# Autodesk Inventor assembly: 217-3433-PTO Config STEP
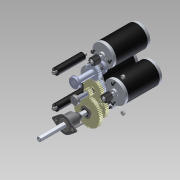
[picture p0: Inventor's stored thumbnail of the model, 180x180]
Saved by Autodesk Inventor 2015 (Build 190159000, 159)
## iProperties
Created: 2015-12-15
Part Number: 217-3433-PTO Config STEP
Document SubType Name: Assembly
Designer: Daniel
Title: 217-3433-PTO Config STEP.STEP
Description: STEP AP214
Creation Date: 2013-12-10
Sending System: SolidWorks 2013
Preprocessor: SwSTEP 2.0
Author: Daniel
## Documents named in this file (45)
- C:\Users\Daniel\Documents\Inventor\West Coast Drive\Imported Components\WCD gear box\217-3433 WCD gear box assembly.iam
- C:\Users\Daniel\Documents\Inventor\West Coast Drive\Imported Components\WCD gear box\217-2428-027 Rev1_97414A630.ipt
- C:\Users\Daniel\Documents\Inventor\West Coast Drive\Imported Components\WCD gear box\217-3423-005 Rev1.ipt
- C:\Users\Daniel\Documents\Inventor\West Coast Drive\Imported Components\WCD gear box\217-3195-200 Rev1.iam
- C:\Users\Daniel\Documents\Inventor\West Coast Drive\Imported Components\WCD gear box\217-3489.ipt
- C:\Users\Daniel\Documents\Inventor\West Coast Drive\Imported Components\WCD gear box\217-3423-006 Rev1.ipt
- C:\Users\Daniel\Documents\Inventor\West Coast Drive\Imported Components\WCD gear box\217-3423-008 Rev1.ipt
- C:\Users\Daniel\Documents\Inventor\West Coast Drive\Imported Components\WCD gear box\217-3423-009 Rev1.ipt
- C:\Users\Daniel\Documents\Inventor\West Coast Drive\Imported Components\WCD gear box\217-2778-001 Rev2_NCQ8A075-050M.iam
- C:\Users\Daniel\Documents\Inventor\West Coast Drive\Imported Components\WCD gear box\217-2731.ipt
- C:\Users\Daniel\Documents\Inventor\West Coast Drive\Imported Components\WCD gear box\217-2733.ipt
- C:\Users\Daniel\Documents\Inventor\West Coast Drive\Imported Components\WCD gear box\217-2734.ipt
- C:\Users\Daniel\Documents\Inventor\West Coast Drive\Imported Components\WCD gear box\217-2743.ipt
- C:\Users\Daniel\Documents\Inventor\West Coast Drive\Imported Components\WCD gear box\217-2614-002_98430A132.ipt
- C:\Users\Daniel\Documents\Inventor\West Coast Drive\Imported Components\WCD gear box\217-3421-007 Rev1.ipt
- C:\Users\Daniel\Documents\Inventor\West Coast Drive\Imported Components\WCD gear box\217-3421-009 Rev1.ipt
- C:\Users\Daniel\Documents\Inventor\West Coast Drive\Imported Components\WCD gear box\217-3421-010 Rev1.ipt
- C:\Users\Daniel\Documents\Inventor\West Coast Drive\Imported Components\WCD gear box\217-3421-011 Rev2_97633A200.ipt
- C:\Users\Daniel\Documents\Inventor\West Coast Drive\Imported Components\WCD gear box\217-3422-007 Rev1.ipt
- C:\Users\Daniel\Documents\Inventor\West Coast Drive\Imported Components\WCD gear box\217-3423-014 Rev1.ipt
- C:\Users\Daniel\Documents\Inventor\West Coast Drive\Imported Components\WCD gear box\217-3423-016 Rev1.ipt
- C:\Users\Daniel\Documents\Inventor\West Coast Drive\Imported Components\WCD gear box\217-3424-003 Rev1.ipt
- C:\Users\Daniel\Documents\Inventor\West Coast Drive\Imported Components\WCD gear box\217-3210-001 Rev1_30t.ipt
- C:\Users\Daniel\Documents\Inventor\West Coast Drive\Imported Components\WCD gear box\217-3215-001 Rev1_42t.ipt
- C:\Users\Daniel\Documents\Inventor\West Coast Drive\Imported Components\WCD gear box\217-3414-001 Rev1_14t Steel Pinion.ipt
- C:\Users\Daniel\Documents\Inventor\West Coast Drive\Imported Components\WCD gear box\217-3418-001 Rev2_44t.ipt
- C:\Users\Daniel\Documents\Inventor\West Coast Drive\Imported Components\WCD gear box\217-3420-001 Rev2_60t.ipt
- C:\Users\Daniel\Documents\Inventor\West Coast Drive\Imported Components\WCD gear box\217-3100-001_14t.ipt
- C:\Users\Daniel\Documents\Inventor\West Coast Drive\Imported Components\WCD gear box\217-2000.ipt
- C:\Users\Daniel\Documents\Inventor\West Coast Drive\Imported Components\WCD gear box\217-3433-001 Rev1_Default_As Machined_.ipt
- C:\Users\Daniel\Documents\Inventor\West Coast Drive\Imported Components\WCD gear box\217-3423-003 Rev1.ipt
- C:\Users\Daniel\Documents\Inventor\West Coast Drive\Imported Components\WCD gear box\217-3424-005 Rev1.ipt
- C:\Users\Daniel\Documents\Inventor\West Coast Drive\Imported Components\WCD gear box\217-3256-001 Rev1.ipt
- C:\Users\Daniel\Documents\Inventor\West Coast Drive\Imported Components\WCD gear box\217-3257-001 Rev1.ipt
- C:\Users\Daniel\Documents\Inventor\West Coast Drive\Imported Components\WCD gear box\217-3259-001 Rev1.ipt
- C:\Users\Daniel\Documents\Inventor\West Coast Drive\Imported Components\WCD gear box\217-3423-004 Rev1.ipt
- C:\Users\Daniel\Documents\Inventor\West Coast Drive\Imported Components\WCD gear box\217-3424-002 Rev1.ipt
- C:\Users\Daniel\Documents\Inventor\West Coast Drive\Imported Components\WCD gear box\217-2758-001 Rev1.ipt
- C:\Users\Daniel\Documents\Inventor\West Coast Drive\Imported Components\WCD gear box\217-3422-004 Rev2.ipt
- C:\Users\Daniel\Documents\Inventor\West Coast Drive\Imported Components\WCD gear box\217-3263-001 Rev1.ipt
- C:\Users\Daniel\Documents\Inventor\West Coast Drive\Imported Components\WCD gear box\217-2761-001 rev1.ipt
- C:\Users\Daniel\Documents\Inventor\West Coast Drive\Imported Components\217-3433-STEP\217-3433-003 Rev1.ipt
- C:\Users\Daniel\Documents\Inventor\West Coast Drive\Imported Components\217-3433-STEP\217-2705-001_30t.ipt
- C:\Users\Daniel\Documents\Inventor\West Coast Drive\Imported Components\217-3433-STEP\217-3261-001 Rev1.ipt
- C:\Users\Daniel\Documents\Inventor\West Coast Drive\Imported Components\217-3433-STEP\217-2731.ipt
## Components (78 placed, 78 different names)
1. 217-2428-027 Rev1_97414A630_1 — Mate:126, Mate:127
2. 217-3423-005 Rev1_2 — Mate:106, Mate:108, Mate:109, Mate:110, Mate:111, Mate:112, Mate:113, Mate:114, Angle:4
3. 217-3195-200 Rev1_3 [sub-assembly] — Mate:128, Angle:6, Mate:129, Mate:130
4. 217-3489_4 — Mate:124, Mate:125, Mate:127, Mate:130
5. 217-3423-006 Rev1_9 — Mate:107, Mate:108
6. 217-3423-006 Rev1_10 — Mate:105, Mate:106, Mate:117
7. 217-3423-008 Rev1_11 — Mate:102, Mate:103, Mate:124, Mate:125, Mate:126, Mate:167
8. 217-3423-009 Rev1_13 — Mate:164, Mate:165, Mate:166, Angle:14
9. 217-2778-001 Rev2_NCQ8A075-050M_16 [sub-assembly] — Mate:113, Mate:114, Angle:4, Mate:128, Angle:6, Mate:129
10. 217-2731_17 — Mate:101, Mate:120, Mate:121, Mate:122, Mate:134, Mate:135, Mate:136
11. 217-2731_18 — Mate:151, Mate:153, Mate:156, Mate:157, Flush:8
12. 217-2733_19 — Flush:7, Mate:140, Mate:148, Mate:149, Mate:150
13. 217-2733_20 — Flush:6, Mate:139
14. 217-2734_21 — Mate:79, Mate:89, Mate:90, Angle:13
15. 217-2734_23 — Mate:91, Mate:92, Mate:93, Mate:94, Angle:2
16. 217-2743_24 — Mate:100, Mate:101, Mate:102, Mate:118, Mate:123, Mate:163
17. 217-2614-002_98430A132_26 — Mate:18, Mate:19
18. 217-2614-002_98430A132_27 — Mate:20, Mate:21
19. 217-2614-002_98430A132_28 — Mate:37, Mate:38
20. 217-2614-002_98430A132_29 — Mate:35, Mate:36
21. 217-2614-002_98430A132_30 — Mate:9, Mate:12
22. 217-2614-002_98430A132_31 — Mate:10, Mate:11
23. 217-3421-007 Rev1_34 — Mate:105, Mate:110, Mate:111, Mate:116
24. 217-3421-007 Rev1_35 — Mate:107, Mate:109, Mate:112, Mate:115
25. 217-3421-009 Rev1_36 — Mate:4, Mate:5
26. 217-3421-009 Rev1_37 — Mate:29, Mate:30
27. 217-3421-009 Rev1_38 — Mate:6, Mate:7
28. 217-3421-009 Rev1_39 — Mate:44, Mate:45
29. 217-3421-009 Rev1_40 — Mate:43, Mate:46
30. 217-3421-009 Rev1_41 — Mate:27, Mate:28
31. 217-3421-010 Rev1_42 — Mate:60, Mate:61
32. 217-3421-010 Rev1_43 — Mate:72, Mate:73
33. 217-3421-010 Rev1_44 — Mate:64, Mate:65
34. 217-3421-010 Rev1_45 — Mate:68, Mate:69
35. 217-3421-011 Rev2_97633A200_47 — Mate:168, Mate:169
36. 217-3422-007 Rev1_48 — Mate:75, Flush:2, Mate:76
37. 217-3422-007 Rev1_49 — Mate:74, Flush:1, Mate:77
38. 217-3423-014 Rev1_50 — Mate:164, Mate:165, Mate:167
39. 217-3423-016 Rev1_52 — Mate:131, Mate:136
40. 217-3423-016 Rev1_53 — Mate:133, Mate:135
41. 217-3423-016 Rev1_54 — Mate:132, Mate:134
42. 217-3424-003 Rev1_55 — Mate:70, Mate:71, Mate:72
43. 217-3424-003 Rev1_56 — Mate:66, Mate:67, Mate:68
44. 217-3424-003 Rev1_57 — Mate:62, Mate:63, Mate:64
45. 217-3424-003 Rev1_58 — Mate:58, Mate:59, Mate:60
46. 217-3210-001 Rev1_30t_59 — Mate:143, Mate:147, Angle:10, Mate:148, Rotation:6
47. 217-3215-001 Rev1_42t_60 — Mate:141, Mate:143, Mate:146, Angle:9, Angle:10, Rotation:2, Rotation:4, Rotation:5
48. 217-3414-001 Rev1_14t Steel Pinion_61 — Mate:34, Mate:36, Mate:37, Mate:39, Rotation:5
49. 217-3414-001 Rev1_14t Steel Pinion_62 — Mate:17, Mate:19, Mate:21, Mate:22, Rotation:4
50. 217-3414-001 Rev1_14t Steel Pinion_63 — Mate:8, Mate:9, Mate:10, Mate:13, Rotation:3
51. 217-3418-001 Rev2_44t_64 — Mate:103, Mate:118, Rotation:6
52. 217-3420-001 Rev2_60t_65 — Mate:91, Mate:92, Mate:96, Angle:14, Angle:15, Rotation:1
53. 217-3100-001_14t_66 — Mate:142, Mate:144, Angle:7, Angle:8, Rotation:1
54. 217-2000_68 — Mate:14, Mate:15, Mate:16, Mate:17, Mate:18, Mate:20, Mate:22, Mate:23, Mate:25, Mate:26
55. 217-2000_69 — Mate:31, Mate:32, Mate:33, Mate:34, Mate:35, Mate:38, Mate:39, Mate:40, Mate:41, Mate:42
56. 217-2000_70 — Mate:1, Mate:2, Mate:3, Mate:8, Mate:11, Mate:12, Mate:13
57. 217-3433-001 Rev1_Default<As Machined>_71 — Mate:1, Mate:2, Mate:3, Mate:4, Mate:5, Mate:6, Mate:7, Mate:23, Mate:25, Mate:26, Mate:27, Mate:28, Mate:29, Mate:30, Mate:40, Mate:41, Mate:42, Mate:43, Mate:44, Mate:45, Mate:46, Mate:47, Mate:48, Mate:49, Mate:50, Mate:51, Mate:52, Mate:53, Mate:54, Mate:61, Mate:65, Mate:69, Mate:73, Mate:88, Mate:115, Mate:116, Mate:117, Mate:120, Mate:121, Mate:131, Mate:132, Mate:133, Mate:149, Mate:150, Mate:154, Mate:155
58. 217-3433-001 Rev1_Default<As Machined>_72 — Mate:55, Mate:56, Mate:57, Mate:58, Mate:59, Mate:63, Mate:67, Mate:71, Mate:76, Mate:77, Mate:78, Mate:151, Mate:156
59. 217-3423-003 Rev1_73 — Mate:87, Angle:1, Mate:88, Mate:96, Mate:163, Mate:166, Mate:168, Mate:169, Angle:13, Angle:15
60. 217-3424-005 Rev1_75 — Flush:6, Mate:139, Flush:7, Mate:140, Mate:144, Mate:145, Mate:146, Mate:147, Angle:7
61. 217-3256-001 Rev1_76 — Mate:141, Mate:142, Mate:145, Angle:8, Angle:9
62. 217-3257-001 Rev1_78 — Mate:93, Mate:94, Angle:2, Mate:95
63. 217-3423-004 Rev1_81 — Mate:100, Mate:122, Mate:123
64. 217-3424-002 Rev1_84 — Mate:49, Mate:50, Mate:66
65. 217-3424-002 Rev1_85 — Mate:52, Mate:54, Mate:56, Mate:70
66. 217-3424-002 Rev1_86 — Mate:47, Mate:48, Mate:62
67. 217-3424-002 Rev1_87 — Mate:51, Mate:53, Mate:55, Mate:57
68. 217-3422-004 Rev2_89 — Mate:74, Flush:1, Mate:75, Flush:2, Mate:78, Mate:79, Mate:90
69. 217-3263-001 Rev1_91 — Mate:81, Mate:82, Mate:83, Mate:86, Flush:3, Mate:87, Angle:1, Mate:89
70. 217-3259-001 Rev1_92 — Mate:81, Mate:85, Mate:86, Flush:3, Flush:4
71. 217-2758-001 Rev1_93 — Mate:83, Mate:84, Flush:5, Mate:95
72. 217-2761-001 rev1_94 — Mate:14, Mate:15, Mate:16
73. 217-2761-001 rev1_95 — Mate:31, Mate:32, Mate:33
74. 217-3257-001 Rev1_100 — Mate:82, Mate:84, Mate:85, Flush:4, Flush:5
75. 217-3433-003 Rev1:1 — Mate:153, Mate:157, Flush:8, Mate:158, Mate:159, Angle:11, Angle:12
76. 217-2705-001_30t:1 — Mate:158, Angle:12, Mate:160, Rotation:2, Rotation:3
77. 217-3261-001 Rev1:1 — Mate:159, Angle:11, Mate:160, Mate:161
78. 217-2731:3 — Mate:154, Mate:155, Mate:161
## Relationships (185: Mate 158, Angle 13, Flush 8, RelateRotation 6)
- Mate:1: 217-2000_70 ↔ 217-3433-001 Rev1_Default<As Machined>_71
- Mate:2: 217-2000_70 ↔ 217-3433-001 Rev1_Default<As Machined>_71
- Mate:3: 217-2000_70 ↔ 217-3433-001 Rev1_Default<As Machined>_71
- Mate:4: 217-3421-009 Rev1_36 ↔ 217-3433-001 Rev1_Default<As Machined>_71
- Mate:5: 217-3421-009 Rev1_36 ↔ 217-3433-001 Rev1_Default<As Machined>_71
- Mate:6: 217-3421-009 Rev1_38 ↔ 217-3433-001 Rev1_Default<As Machined>_71
- Mate:7: 217-3421-009 Rev1_38 ↔ 217-3433-001 Rev1_Default<As Machined>_71
- Mate:8: 217-3414-001 Rev1_14t Steel Pinion_63 ↔ 217-2000_70
- Mate:9: 217-2614-002_98430A132_30 ↔ 217-3414-001 Rev1_14t Steel Pinion_63
- Mate:10: 217-2614-002_98430A132_31 ↔ 217-3414-001 Rev1_14t Steel Pinion_63
- Mate:11: 217-2614-002_98430A132_31 ↔ 217-2000_70
- Mate:12: 217-2614-002_98430A132_30 ↔ 217-2000_70
- Mate:13 (10.2113 mm): 217-3414-001 Rev1_14t Steel Pinion_63 ↔ 217-2000_70
- Mate:14: 217-2000_68 ↔ 217-2761-001 rev1_94
- Mate:15: 217-2000_68 ↔ 217-2761-001 rev1_94
- Mate:16: 217-2000_68 ↔ 217-2761-001 rev1_94
- Mate:17: 217-3414-001 Rev1_14t Steel Pinion_62 ↔ 217-2000_68
- Mate:18: 217-2614-002_98430A132_26 ↔ 217-2000_68
- Mate:19: 217-2614-002_98430A132_26 ↔ 217-3414-001 Rev1_14t Steel Pinion_62
- Mate:20: 217-2614-002_98430A132_27 ↔ 217-2000_68
- Mate:21: 217-2614-002_98430A132_27 ↔ 217-3414-001 Rev1_14t Steel Pinion_62
- Mate:22 (10.2113 mm): 217-3414-001 Rev1_14t Steel Pinion_62 ↔ 217-2000_68
- Mate:23: 217-2000_68 ↔ 217-3433-001 Rev1_Default<As Machined>_71
- Mate:25: 217-2000_68 ↔ 217-3433-001 Rev1_Default<As Machined>_71
- Mate:26: 217-2000_68 ↔ 217-3433-001 Rev1_Default<As Machined>_71
- Mate:27: 217-3421-009 Rev1_41 ↔ 217-3433-001 Rev1_Default<As Machined>_71
- Mate:28: 217-3421-009 Rev1_41 ↔ 217-3433-001 Rev1_Default<As Machined>_71
- Mate:29: 217-3421-009 Rev1_37 ↔ 217-3433-001 Rev1_Default<As Machined>_71
- Mate:30: 217-3421-009 Rev1_37 ↔ 217-3433-001 Rev1_Default<As Machined>_71
- Mate:31: 217-2000_69 ↔ 217-2761-001 rev1_95
- Mate:32: 217-2000_69 ↔ 217-2761-001 rev1_95
- Mate:33: 217-2000_69 ↔ 217-2761-001 rev1_95
- Mate:34: 217-3414-001 Rev1_14t Steel Pinion_61 ↔ 217-2000_69
- Mate:35: 217-2614-002_98430A132_29 ↔ 217-2000_69
- Mate:36: 217-2614-002_98430A132_29 ↔ 217-3414-001 Rev1_14t Steel Pinion_61
- Mate:37: 217-2614-002_98430A132_28 ↔ 217-3414-001 Rev1_14t Steel Pinion_61
- Mate:38: 217-2614-002_98430A132_28 ↔ 217-2000_69
- Mate:39 (10.2113 mm): 217-3414-001 Rev1_14t Steel Pinion_61 ↔ 217-2000_69
- Mate:40: 217-2000_69 ↔ 217-3433-001 Rev1_Default<As Machined>_71
- Mate:41: 217-2000_69 ↔ 217-3433-001 Rev1_Default<As Machined>_71
- Mate:42: 217-2000_69 ↔ 217-3433-001 Rev1_Default<As Machined>_71
- Mate:43: 217-3421-009 Rev1_40 ↔ 217-3433-001 Rev1_Default<As Machined>_71
- Mate:44: 217-3421-009 Rev1_39 ↔ 217-3433-001 Rev1_Default<As Machined>_71
- Mate:45: 217-3421-009 Rev1_39 ↔ 217-3433-001 Rev1_Default<As Machined>_71
- Mate:46: 217-3421-009 Rev1_40 ↔ 217-3433-001 Rev1_Default<As Machined>_71
- Mate:47: 217-3433-001 Rev1_Default<As Machined>_71 ↔ 217-3424-002 Rev1_86
- Mate:48: 217-3433-001 Rev1_Default<As Machined>_71 ↔ 217-3424-002 Rev1_86
- Mate:49: 217-3433-001 Rev1_Default<As Machined>_71 ↔ 217-3424-002 Rev1_84
- Mate:50: 217-3433-001 Rev1_Default<As Machined>_71 ↔ 217-3424-002 Rev1_84
- Mate:51: 217-3433-001 Rev1_Default<As Machined>_71 ↔ 217-3424-002 Rev1_87
- Mate:52: 217-3433-001 Rev1_Default<As Machined>_71 ↔ 217-3424-002 Rev1_85
- Mate:53: 217-3433-001 Rev1_Default<As Machined>_71 ↔ 217-3424-002 Rev1_87
- Mate:54: 217-3433-001 Rev1_Default<As Machined>_71 ↔ 217-3424-002 Rev1_85
- Mate:55: 217-3433-001 Rev1_Default<As Machined>_72 ↔ 217-3424-002 Rev1_87
- Mate:56: 217-3433-001 Rev1_Default<As Machined>_72 ↔ 217-3424-002 Rev1_85
- Mate:57: 217-3433-001 Rev1_Default<As Machined>_72 ↔ 217-3424-002 Rev1_87
- Mate:58: 217-3424-003 Rev1_58 ↔ 217-3433-001 Rev1_Default<As Machined>_72
- Mate:59: 217-3424-003 Rev1_58 ↔ 217-3433-001 Rev1_Default<As Machined>_72
- Mate:60: 217-3421-010 Rev1_42 ↔ 217-3424-003 Rev1_58
- Mate:61: 217-3421-010 Rev1_42 ↔ 217-3433-001 Rev1_Default<As Machined>_71
- Mate:62: 217-3424-003 Rev1_57 ↔ 217-3424-002 Rev1_86
- Mate:63: 217-3424-003 Rev1_57 ↔ 217-3433-001 Rev1_Default<As Machined>_72
- Mate:64: 217-3421-010 Rev1_44 ↔ 217-3424-003 Rev1_57
- Mate:65: 217-3421-010 Rev1_44 ↔ 217-3433-001 Rev1_Default<As Machined>_71
- Mate:66: 217-3424-003 Rev1_56 ↔ 217-3424-002 Rev1_84
- Mate:67: 217-3424-003 Rev1_56 ↔ 217-3433-001 Rev1_Default<As Machined>_72
- Mate:68: 217-3421-010 Rev1_45 ↔ 217-3424-003 Rev1_56
- Mate:69: 217-3421-010 Rev1_45 ↔ 217-3433-001 Rev1_Default<As Machined>_71
- Mate:70: 217-3424-003 Rev1_55 ↔ 217-3424-002 Rev1_85
- Mate:71: 217-3424-003 Rev1_55 ↔ 217-3433-001 Rev1_Default<As Machined>_72
- Mate:72: 217-3421-010 Rev1_43 ↔ 217-3424-003 Rev1_55
- Mate:73: 217-3421-010 Rev1_43 ↔ 217-3433-001 Rev1_Default<As Machined>_71
- Mate:74: 217-3422-007 Rev1_49 ↔ 217-3422-004 Rev2_89
- Flush:1: 217-3422-007 Rev1_49 ↔ 217-3422-004 Rev2_89
- Mate:75: 217-3422-007 Rev1_48 ↔ 217-3422-004 Rev2_89
- Flush:2: 217-3422-007 Rev1_48 ↔ 217-3422-004 Rev2_89
- Mate:76: 217-3422-007 Rev1_48 ↔ 217-3433-001 Rev1_Default<As Machined>_72
- Mate:77: 217-3422-007 Rev1_49 ↔ 217-3433-001 Rev1_Default<As Machined>_72
- Mate:78: 217-3433-001 Rev1_Default<As Machined>_72 ↔ 217-3422-004 Rev2_89
- Mate:79: 217-2734_21 ↔ 217-3422-004 Rev2_89
- Mate:81: 217-3263-001 Rev1_91 ↔ 217-3259-001 Rev1_92
- Mate:82: 217-3263-001 Rev1_91 ↔ 217-3257-001 Rev1_100
- Mate:83: 217-3263-001 Rev1_91 ↔ 217-2758-001 Rev1_93
- Mate:84: 217-2758-001 Rev1_93 ↔ 217-3257-001 Rev1_100
- Mate:85: 217-3259-001 Rev1_92 ↔ 217-3257-001 Rev1_100
- Mate:86: 217-3263-001 Rev1_91 ↔ 217-3259-001 Rev1_92
- Flush:3: 217-3263-001 Rev1_91 ↔ 217-3259-001 Rev1_92
- Flush:4: 217-3259-001 Rev1_92 ↔ 217-3257-001 Rev1_100
- Flush:5: 217-2758-001 Rev1_93 ↔ 217-3257-001 Rev1_100
- Mate:87: 217-3423-003 Rev1_73 ↔ 217-3263-001 Rev1_91
- Angle:1 (0 deg): 217-3423-003 Rev1_73 ↔ 217-3263-001 Rev1_91
- Mate:88: 217-3433-001 Rev1_Default<As Machined>_71 ↔ 217-3423-003 Rev1_73
- Mate:89: 217-2734_21 ↔ 217-3263-001 Rev1_91
- Mate:90: 217-2734_21 ↔ 217-3422-004 Rev2_89
- Mate:91: 217-2734_23 ↔ 217-3420-001 Rev2_60t_65
- Mate:92: 217-2734_23 ↔ 217-3420-001 Rev2_60t_65
- Mate:93: 217-2734_23 ↔ 217-3257-001 Rev1_78
- Mate:94: 217-2734_23 ↔ 217-3257-001 Rev1_78
- Angle:2 (0 deg): 217-2734_23 ↔ 217-3257-001 Rev1_78
- Mate:95 (18.3389 mm): 217-3257-001 Rev1_78 ↔ 217-2758-001 Rev1_93
- Mate:96: 217-3420-001 Rev2_60t_65 ↔ 217-3423-003 Rev1_73
- Mate:100: 217-2743_24 ↔ 217-3423-004 Rev1_81
- Mate:101: 217-2731_17 ↔ 217-2743_24
- Mate:102: 217-3423-008 Rev1_11 ↔ 217-2743_24
- Mate:103: 217-3423-008 Rev1_11 ↔ 217-3418-001 Rev2_44t_64
- Mate:105: 217-3423-006 Rev1_10 ↔ 217-3421-007 Rev1_34
- Mate:106: 217-3423-005 Rev1_2 ↔ 217-3423-006 Rev1_10
- Mate:107: 217-3423-006 Rev1_9 ↔ 217-3421-007 Rev1_35
- Mate:108: 217-3423-005 Rev1_2 ↔ 217-3423-006 Rev1_9
- Mate:109: 217-3423-005 Rev1_2 ↔ 217-3421-007 Rev1_35
- Mate:110: 217-3423-005 Rev1_2 ↔ 217-3421-007 Rev1_34
- Mate:111: 217-3423-005 Rev1_2 ↔ 217-3421-007 Rev1_34
- Mate:112: 217-3423-005 Rev1_2 ↔ 217-3421-007 Rev1_35
- Mate:113: 217-3423-005 Rev1_2 ↔ 217-2778-001 Rev2_NCQ8A075-050M_16
- Mate:114: 217-3423-005 Rev1_2 ↔ 217-2778-001 Rev2_NCQ8A075-050M_16
- Mate:115: 217-3421-007 Rev1_35 ↔ 217-3433-001 Rev1_Default<As Machined>_71
- Mate:116: 217-3421-007 Rev1_34 ↔ 217-3433-001 Rev1_Default<As Machined>_71
- Mate:117: 217-3423-006 Rev1_10 ↔ 217-3433-001 Rev1_Default<As Machined>_71
- Angle:4 (1.1459 deg): 217-3423-005 Rev1_2 ↔ 217-2778-001 Rev2_NCQ8A075-050M_16
- Mate:118: 217-2743_24 ↔ 217-3418-001 Rev2_44t_64
- Mate:120: 217-2731_17 ↔ 217-3433-001 Rev1_Default<As Machined>_71
- Mate:121: 217-2731_17 ↔ 217-3433-001 Rev1_Default<As Machined>_71
- Mate:122: 217-2731_17 ↔ 217-3423-004 Rev1_81
- Mate:123: 217-2743_24 ↔ 217-3423-004 Rev1_81
- Mate:124: 217-3489_4 ↔ 217-3423-008 Rev1_11
- Mate:125: 217-3489_4 ↔ 217-3423-008 Rev1_11
- Mate:126: 217-2428-027 Rev1_97414A630_1 ↔ 217-3423-008 Rev1_11
- Mate:127: 217-2428-027 Rev1_97414A630_1 ↔ 217-3489_4
- Mate:128: 217-3195-200 Rev1_3 ↔ 217-2778-001 Rev2_NCQ8A075-050M_16
- Angle:6 (180 deg): 217-3195-200 Rev1_3 ↔ 217-2778-001 Rev2_NCQ8A075-050M_16
- Mate:129: 217-3195-200 Rev1_3 ↔ 217-2778-001 Rev2_NCQ8A075-050M_16
- Mate:130: 217-3195-200 Rev1_3 ↔ 217-3489_4
- Mate:131: 217-3423-016 Rev1_52 ↔ 217-3433-001 Rev1_Default<As Machined>_71
- Mate:132: 217-3423-016 Rev1_54 ↔ 217-3433-001 Rev1_Default<As Machined>_71
- Mate:133: 217-3423-016 Rev1_53 ↔ 217-3433-001 Rev1_Default<As Machined>_71
- Mate:134: 217-2731_17 ↔ 217-3423-016 Rev1_54
- Mate:135: 217-2731_17 ↔ 217-3423-016 Rev1_53
- Mate:136: 217-2731_17 ↔ 217-3423-016 Rev1_52
- Flush:6: 217-2733_20 ↔ 217-3424-005 Rev1_75
- Mate:139: 217-2733_20 ↔ 217-3424-005 Rev1_75
- Flush:7: 217-2733_19 ↔ 217-3424-005 Rev1_75
- Mate:140: 217-2733_19 ↔ 217-3424-005 Rev1_75
- Mate:141: 217-3215-001 Rev1_42t_60 ↔ 217-3256-001 Rev1_76
- Mate:142: 217-3100-001_14t_66 ↔ 217-3256-001 Rev1_76
- Mate:143: 217-3210-001 Rev1_30t_59 ↔ 217-3215-001 Rev1_42t_60
- Mate:144: 217-3100-001_14t_66 ↔ 217-3424-005 Rev1_75
- Mate:145: 217-3424-005 Rev1_75 ↔ 217-3256-001 Rev1_76
- Mate:146: 217-3215-001 Rev1_42t_60 ↔ 217-3424-005 Rev1_75
- Mate:147: 217-3210-001 Rev1_30t_59 ↔ 217-3424-005 Rev1_75
- Angle:7 (0 deg): 217-3100-001_14t_66 ↔ 217-3424-005 Rev1_75
- Angle:8 (0 deg): 217-3100-001_14t_66 ↔ 217-3256-001 Rev1_76
- Angle:9 (0 deg): 217-3215-001 Rev1_42t_60 ↔ 217-3256-001 Rev1_76
- Angle:10 (0 deg): 217-3210-001 Rev1_30t_59 ↔ 217-3215-001 Rev1_42t_60
- Mate:148: 217-2733_19 ↔ 217-3210-001 Rev1_30t_59
- Mate:149: 217-2733_19 ↔ 217-3433-001 Rev1_Default<As Machined>_71
- Mate:150: 217-2733_19 ↔ 217-3433-001 Rev1_Default<As Machined>_71
- Mate:151: 217-2731_18 ↔ 217-3433-001 Rev1_Default<As Machined>_72
- Mate:153: 217-2731_18 ↔ 217-3433-003 Rev1:1
- Mate:154: 217-3433-001 Rev1_Default<As Machined>_71 ↔ 217-2731:3
- Mate:155: 217-3433-001 Rev1_Default<As Machined>_71 ↔ 217-2731:3
- Mate:156: 217-2731_18 ↔ 217-3433-001 Rev1_Default<As Machined>_72
- Mate:157: 217-2731_18 ↔ 217-3433-003 Rev1:1
- Flush:8: 217-2731_18 ↔ 217-3433-003 Rev1:1
- Mate:158: 217-3433-003 Rev1:1 ↔ 217-2705-001_30t:1
- Mate:159: 217-3433-003 Rev1:1 ↔ 217-3261-001 Rev1:1
- Angle:11 (0 deg): 217-3433-003 Rev1:1 ↔ 217-3261-001 Rev1:1
- Angle:12 (0 deg): 217-3433-003 Rev1:1 ↔ 217-2705-001_30t:1
- Mate:160: 217-2705-001_30t:1 ↔ 217-3261-001 Rev1:1
- Mate:161: 217-3261-001 Rev1:1 ↔ 217-2731:3
- Mate:163: 217-2743_24 ↔ 217-3423-003 Rev1_73
- Mate:164: 217-3423-009 Rev1_13 ↔ 217-3423-014 Rev1_50
- Mate:165: 217-3423-009 Rev1_13 ↔ 217-3423-014 Rev1_50
- Mate:166: 217-3423-009 Rev1_13 ↔ 217-3423-003 Rev1_73
- Mate:167: 217-3423-008 Rev1_11 ↔ 217-3423-014 Rev1_50
- Mate:168: 217-3421-011 Rev2_97633A200_47 ↔ 217-3423-003 Rev1_73
- Mate:169: 217-3421-011 Rev2_97633A200_47 ↔ 217-3423-003 Rev1_73
- Angle:13 (0 deg): 217-2734_21 ↔ 217-3423-003 Rev1_73
- Angle:14 (0 deg): 217-3423-009 Rev1_13 ↔ 217-3420-001 Rev2_60t_65
- Angle:15 (0 deg): 217-3420-001 Rev2_60t_65 ↔ 217-3423-003 Rev1_73
- Rotation:1 [RelateRotation] (3.875 ul): 217-3420-001 Rev2_60t_65 ↔ 217-3100-001_14t_66
- Rotation:2 [RelateRotation] (1.375 ul): 217-3215-001 Rev1_42t_60 ↔ 217-2705-001_30t:1
- Rotation:3 [RelateRotation] (2 ul): 217-3414-001 Rev1_14t Steel Pinion_63 ↔ 217-2705-001_30t:1
- Rotation:4 [RelateRotation] (2.75 ul): 217-3215-001 Rev1_42t_60 ↔ 217-3414-001 Rev1_14t Steel Pinion_62
- Rotation:5 [RelateRotation] (0.364 ul): 217-3215-001 Rev1_42t_60 ↔ 217-3414-001 Rev1_14t Steel Pinion_61
- Rotation:6 [RelateRotation] (1.438 ul): 217-3210-001 Rev1_30t_59 ↔ 217-3418-001 Rev2_44t_64
